# Autodesk Inventor assembly: bellows_latest
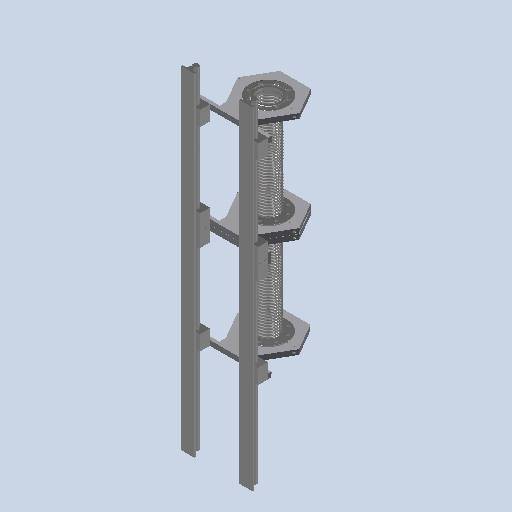
[picture p0: Inventor's stored thumbnail of the model, 512x512]
Saved by Autodesk Inventor 2026.3 (Build 303398000, 398)
## iProperties
Created: 2026-06-04
Part Number: bellows_latest
Document SubType Name: Assembly
Designer: shusu
Author: shusu
## Documents named in this file (3)
- C:\Users\shusu\aklab_pihti\PIHTI\bellows\bellows.iam
- C:\Users\shusu\aklab_pihti\PIHTI\bellows\bellows_1.iam
- C:\Users\shusu\aklab_pihti\PIHTI\bellows\rail.ipt
## Components (4 placed, 2 different names)
1. bellows_1:1 [sub-assembly] — メイト:1, 角度:1, 角度:2, 挿入:1, 挿入:2
2. bellows_1:2 [sub-assembly] — メイト:1
3. rail:1 — 角度:1, 挿入:1
4. rail:2 — 角度:2, 挿入:2
## Relationships (5: Angle 2, Insert 2, Mate 1)
- メイト:1 [Mate]: bellows_1:1 ↔ bellows_1:2
- 角度:1 [Angle] (0 deg): bellows_1:1 ↔ rail:1
- 角度:2 [Angle] (0 deg): bellows_1:1 ↔ rail:2
- 挿入:1 [Insert] (-100 mm): bellows_1:1 ↔ rail:1
- 挿入:2 [Insert] (-100 mm): bellows_1:1 ↔ rail:2
